# Autodesk Inventor assembly: 3rd_floor
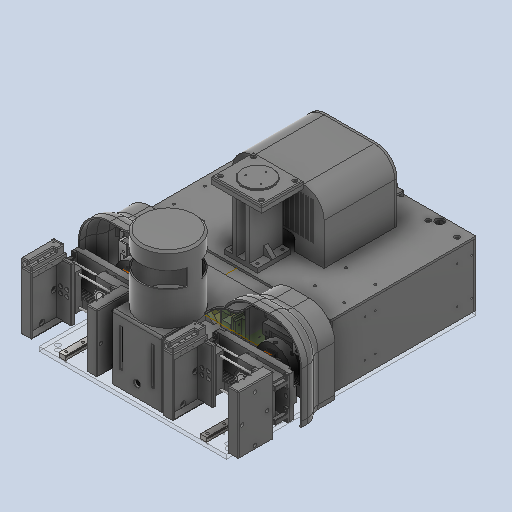
[picture p0: Inventor's stored thumbnail of the model, 512x512]
Saved by Autodesk Inventor 2026.2 (Build 302298010, 298A)
## iProperties
Created: 2026-05-16
Part Number: 3rd_floor
Document SubType Name: Assembly
Designer: chris
Author: chris
## Documents named in this file (11)
- C:\Users\chanh\내 드라이브\교과공부\2026년 1학기 (4학년 1학기)\01창의제품설계\UMMA_CAD\04그리퍼\3rd_floor.iam
- C:\Users\chanh\내 드라이브\교과공부\2026년 1학기 (4학년 1학기)\01창의제품설계\UMMA_CAD\04그리퍼\acrilic\acrylic_assemble.iam
- C:\Users\chanh\내 드라이브\교과공부\2026년 1학기 (4학년 1학기)\01창의제품설계\UMMA_CAD\04그리퍼\gripper\gripper.iam
- C:\Users\chanh\내 드라이브\교과공부\2026년 1학기 (4학년 1학기)\01창의제품설계\UMMA_CAD\04그리퍼\addition\gripper_case\gripper_case_front.ipt
- C:\Users\chanh\내 드라이브\교과공부\2026년 1학기 (4학년 1학기)\01창의제품설계\UMMA_CAD\04그리퍼\addition\gripper_case\gripper_case_bracket.ipt
- C:\Users\chanh\내 드라이브\교과공부\2026년 1학기 (4학년 1학기)\01창의제품설계\UMMA_CAD\04그리퍼\addition\gripper_case\gripper_case_upper.ipt
- C:\Users\chanh\내 드라이브\교과공부\2026년 1학기 (4학년 1학기)\01창의제품설계\UMMA_CAD\04그리퍼\addition\gripper_case\gripper_case_upper2.ipt
- C:\Users\chanh\내 드라이브\교과공부\2026년 1학기 (4학년 1학기)\01창의제품설계\UMMA_CAD\04그리퍼\addition\siren_camera\siren_new.ipt
- C:\Users\chanh\내 드라이브\교과공부\2026년 1학기 (4학년 1학기)\01창의제품설계\UMMA_CAD\04그리퍼\addition\siren_camera\speaker.ipt
- C:\Users\chanh\내 드라이브\교과공부\2026년 1학기 (4학년 1학기)\01창의제품설계\UMMA_CAD\04그리퍼\addition\siren_camera\speaker_front.ipt
- C:\Users\chanh\내 드라이브\교과공부\2026년 1학기 (4학년 1학기)\01창의제품설계\UMMA_CAD\04그리퍼\addition\switch\Part1.ipt
## Components (12 placed, 10 different names)
1. acrylic_assemble:1 [sub-assembly] — Flush:1, Flush:2, Flush:3, Mate:3, Mate:4, Mate:5, Mate:6, Rigid:1, Rigid:7, Mate:8
2. gripper:2 [sub-assembly] — Mate:3, Mate:4, Rigid:3
3. gripper:3 [sub-assembly] — Mate:5, Mate:6, Rigid:2
4. gripper_case_front:1 — Rigid:1, Mate:7, Angle:1, Insert:1
5. gripper_case_bracket:1 — Rigid:2, Rigid:4
6. gripper_case_bracket:2 — Rigid:3, Rigid:5
7. gripper_case_upper:1 — Rigid:4
8. gripper_case_upper2:1 — Rigid:5
9. siren_new:1 — Mate:7, Angle:1, Insert:1
10. speaker:1 — Rigid:6, Rigid:7
11. speaker_front:1 — Rigid:6, Flush:4, Mate:9
12. Part1:1 — Flush:4, Mate:8, Mate:9
## Relationships (20: Mate 7, WeldJoint 7, Flush 4, Angle 1, Insert 1)
- Flush:1: acrylic_assemble:1
- Flush:2: acrylic_assemble:1
- Flush:3: acrylic_assemble:1
- Mate:3: acrylic_assemble:1 ↔ gripper:2
- Mate:4: acrylic_assemble:1 ↔ gripper:2
- Mate:5: acrylic_assemble:1 ↔ gripper:3
- Mate:6: acrylic_assemble:1 ↔ gripper:3
- Rigid:1 [WeldJoint]: acrylic_assemble:1 ↔ gripper_case_front:1
- Rigid:2 [WeldJoint]: gripper:3 ↔ gripper_case_bracket:1
- Rigid:3 [WeldJoint]: gripper:2 ↔ gripper_case_bracket:2
- Rigid:4 [WeldJoint]: gripper_case_bracket:1 ↔ gripper_case_upper:1
- Rigid:5 [WeldJoint]: gripper_case_bracket:2 ↔ gripper_case_upper2:1
- Mate:7: gripper_case_front:1 ↔ siren_new:1
- Angle:1 (105 deg): gripper_case_front:1 ↔ siren_new:1
- Insert:1: gripper_case_front:1 ↔ siren_new:1
- Rigid:6 [WeldJoint]: speaker:1 ↔ speaker_front:1
- Rigid:7 [WeldJoint]: acrylic_assemble:1 ↔ speaker:1
- Flush:4: speaker_front:1 ↔ Part1:1
- Mate:8: acrylic_assemble:1 ↔ Part1:1
- Mate:9: speaker_front:1 ↔ Part1:1
